# Autodesk Inventor assembly: Assembly_Cube_Z-Focus_Linearbearing_mechanical_1x1_v3
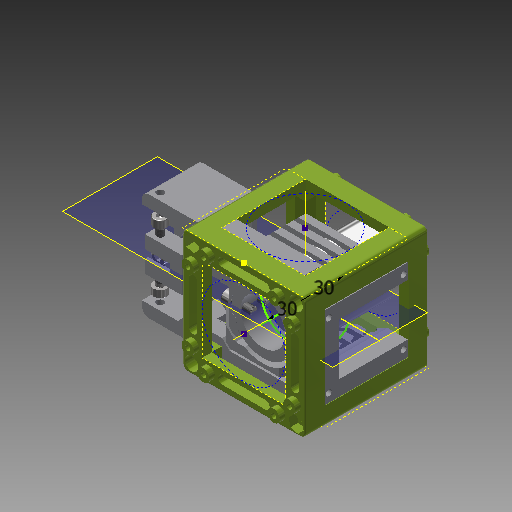
[picture p0: Inventor's stored thumbnail of the model, 512x512]
Saved by Autodesk Inventor 2019 (Build 230136000, 136)
## iProperties
Created: 2020-07-30
Part Number: Assembly_Cube_Z-Focus_Linearbearing_mechanical_1x1_v3
Document SubType Name: Assembly
Designer: marsikovabarbora
Author: marsikovabarbora
## Documents named in this file (9)
- C:\Users\marsikovabarbora\Dropbox\UC2\02_CAD\INVENTOR\uc2_v3\Assembly_Cube_Z-Focus_Linearbearing_mechanical_1x1_v3.iam
- C:\Users\marsikovabarbora\Dropbox\UC2\02_CAD\INVENTOR\uc2_v3\Assembly_Cube_empty_IM_v3.iam
- C:\Users\marsikovabarbora\Dropbox\UC2\02_CAD\INVENTOR\uc2_v3\20_focus_inlet_linearflexure_mechanical_v3.ipt
- C:\Users\marsikovabarbora\Dropbox\UC2\02_CAD\INVENTOR\uc2_v3\20_gear.ipt
- C:\Users\marsikovabarbora\Documents\Inventor\Content Center Files\R2019\en-US\DIN 912\DIN 912 - M3 x 0,5 x 30 x 18.ipt
- C:\Users\marsikovabarbora\Documents\Inventor\Content Center Files\R2019\en-US\DIN 912\DIN 912 - M3 x 0,5 x 8 x 6,75.ipt
- C:\Users\marsikovabarbora\Dropbox\UC2\02_CAD\INVENTOR\uc2_v3\20_focus_inlet_objective_mount_v8.ipt
- C:\Users\marsikovabarbora\Dropbox\UC2\02_CAD\INVENTOR\uc2_v3\00_Microscope_Objective_Lens10x.ipt
- C:\Users\marsikovabarbora\Documents\Inventor\Content Center Files\R2019\en-US\DIN 934\DIN 934 - M3 x 0,5.ipt
## Components (11 placed, 8 different names)
1. Assembly_Cube_empty_IM_v3:1 [sub-assembly] — Mate:1, Mate:2, Flush:1, Mate:27, Flush:5, Flush:6
2. 20_focus_inlet_linearflexure_mechanical_v3:1 — Mate:8, Mate:11, Mate:13, Mate:14, Mate:15, Mate:16, Passend:21, Passend:23, Fluchtend:3, Passend:26, Mate:27, Flush:5, Flush:6
3. 20_gear:1 — Mate:13, Passend:24, Fluchtend:4, Passend:26
4. DIN 912 - replaced by DIN EN ISO 4762 M3 x 30:1 — Mate:11, Mate:14, Tangent:1, Tangent:2, Passend:25
5. DIN 912 - replaced by DIN EN ISO 4762 M3 x 8:1 — Mate:15, Tangent:2
6. DIN 912 - replaced by DIN EN ISO 4762 M3 x 8:2 — Mate:16, Tangent:1
7. DIN 912 - replaced by DIN EN ISO 4762 M3 x 8:3 — Mate:8, Passend:19, Fluchtend:2
8. 20_focus_inlet_objective_mount_v8:1 — Mate:18, Passend:19, Passend:20, Passend:21, Passend:22, Fluchtend:3
9. 00_Microscope_Objective_Lens10x:1 — Mate:18, Passend:22
10. DIN 912 - replaced by DIN EN ISO 4762 M3 x 8:5 — Passend:20, Fluchtend:2, Passend:23
11. DIN 934 - replaced by DIN EN 24032/28673/28674 M3:1 — Passend:24, Fluchtend:4, Passend:25
## Relationships (26: Mate 18, Flush 6, Tangent 2)
- Mate:1: Assembly_Cube_empty_IM_v3:1
- Mate:2: Assembly_Cube_empty_IM_v3:1
- Flush:1: Assembly_Cube_empty_IM_v3:1
- Mate:8: 20_focus_inlet_linearflexure_mechanical_v3:1 ↔ DIN 912 - replaced by DIN EN ISO 4762 M3 x 8:3
- Mate:11: 20_focus_inlet_linearflexure_mechanical_v3:1 ↔ DIN 912 - replaced by DIN EN ISO 4762 M3 x 30:1
- Mate:13: 20_focus_inlet_linearflexure_mechanical_v3:1 ↔ 20_gear:1
- Mate:14: 20_focus_inlet_linearflexure_mechanical_v3:1 ↔ DIN 912 - replaced by DIN EN ISO 4762 M3 x 30:1
- Mate:15: 20_focus_inlet_linearflexure_mechanical_v3:1 ↔ DIN 912 - replaced by DIN EN ISO 4762 M3 x 8:1
- Mate:16: 20_focus_inlet_linearflexure_mechanical_v3:1 ↔ DIN 912 - replaced by DIN EN ISO 4762 M3 x 8:2
- Tangent:1: DIN 912 - replaced by DIN EN ISO 4762 M3 x 30:1 ↔ DIN 912 - replaced by DIN EN ISO 4762 M3 x 8:2
- Tangent:2: DIN 912 - replaced by DIN EN ISO 4762 M3 x 30:1 ↔ DIN 912 - replaced by DIN EN ISO 4762 M3 x 8:1
- Mate:18: 20_focus_inlet_objective_mount_v8:1 ↔ 00_Microscope_Objective_Lens10x:1
- Passend:19 [Mate]: DIN 912 - replaced by DIN EN ISO 4762 M3 x 8:3 ↔ 20_focus_inlet_objective_mount_v8:1
- Passend:20 [Mate]: 20_focus_inlet_objective_mount_v8:1 ↔ DIN 912 - replaced by DIN EN ISO 4762 M3 x 8:5
- Fluchtend:2 [Flush]: DIN 912 - replaced by DIN EN ISO 4762 M3 x 8:3 ↔ DIN 912 - replaced by DIN EN ISO 4762 M3 x 8:5
- Passend:21 [Mate]: 20_focus_inlet_linearflexure_mechanical_v3:1 ↔ 20_focus_inlet_objective_mount_v8:1
- Passend:22 [Mate]: 20_focus_inlet_objective_mount_v8:1 ↔ 00_Microscope_Objective_Lens10x:1
- Passend:23 [Mate]: 20_focus_inlet_linearflexure_mechanical_v3:1 ↔ DIN 912 - replaced by DIN EN ISO 4762 M3 x 8:5
- Fluchtend:3 [Flush]: 20_focus_inlet_linearflexure_mechanical_v3:1 ↔ 20_focus_inlet_objective_mount_v8:1
- Passend:24 [Mate]: 20_gear:1 ↔ DIN 934 - replaced by DIN EN 24032/28673/28674 M3:1
- Fluchtend:4 [Flush]: 20_gear:1 ↔ DIN 934 - replaced by DIN EN 24032/28673/28674 M3:1
- Passend:25 [Mate]: DIN 912 - replaced by DIN EN ISO 4762 M3 x 30:1 ↔ DIN 934 - replaced by DIN EN 24032/28673/28674 M3:1
- Passend:26 [Mate]: 20_focus_inlet_linearflexure_mechanical_v3:1 ↔ 20_gear:1
- Mate:27: Assembly_Cube_empty_IM_v3:1 ↔ 20_focus_inlet_linearflexure_mechanical_v3:1
- Flush:5: Assembly_Cube_empty_IM_v3:1 ↔ 20_focus_inlet_linearflexure_mechanical_v3:1
- Flush:6: Assembly_Cube_empty_IM_v3:1 ↔ 20_focus_inlet_linearflexure_mechanical_v3:1
